# Autodesk Inventor assembly: 32 spocket with hub
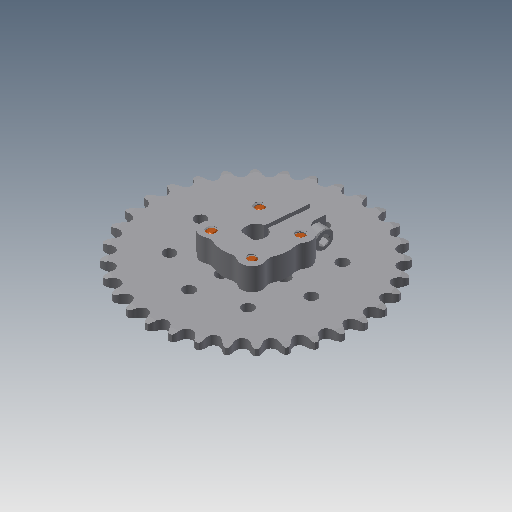
[picture p0: Inventor's stored thumbnail of the model, 512x512]
Saved by Autodesk Inventor 2019 (Build 230136000, 136)
## iProperties
Created: 2019-09-29
Part Number: 32 spocket with hub
Document SubType Name: Assembly
Designer: ball
Author: ball
## Documents named in this file (4)
- C:\FTC\FTC8863CAD\2019 Robot\Mecanum Drive Train\32 spocket with hub.iam
- C:\FTC\FTC8863CAD\Actobotics\545 parts\545618 assembly.ipt
- C:\FTC\FTC8863CAD\Actobotics\615 parts\615114.ipt
- C:\FTC\FTC8863CAD\Actobotics\632 parts\632110.ipt
## Components (6 placed, 3 different names)
1. 545618 assembly:1 — Mate:1, Mate:2, Mate:3, Mate:4, Mate:6
2. 615114:1 — Mate:1, Mate:2, Mate:3, Mate:5, Mate:7, Mate:8, Mate:9, Mate:10, Mate:11
3. 632110:1 — Mate:4, Mate:5
4. 632110:5 — Mate:6, Mate:7
5. 632110:6 — Mate:8, Mate:11
6. 632110:7 — Mate:9, Mate:10
## Relationships (11: Mate 11)
- Mate:1: 545618 assembly:1 ↔ 615114:1
- Mate:2: 545618 assembly:1 ↔ 615114:1
- Mate:3: 545618 assembly:1 ↔ 615114:1
- Mate:4: 545618 assembly:1 ↔ 632110:1
- Mate:5: 615114:1 ↔ 632110:1
- Mate:6: 545618 assembly:1 ↔ 632110:5
- Mate:7: 615114:1 ↔ 632110:5
- Mate:8: 615114:1 ↔ 632110:6
- Mate:9: 615114:1 ↔ 632110:7
- Mate:10: 615114:1 ↔ 632110:7
- Mate:11: 615114:1 ↔ 632110:6
